# Autodesk Inventor assembly: Extruder Assembly
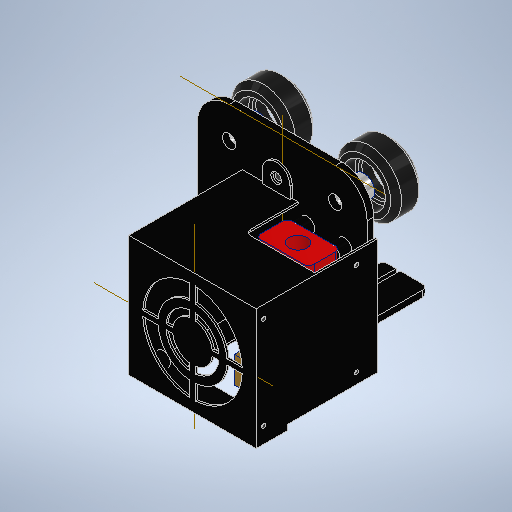
[picture p0: Inventor's stored thumbnail of the model, 512x512]
Saved by Autodesk Inventor 2025.2 (Build 292293000, 293)
## iProperties
Created: 2025-03-12
Part Number: Extruder Assembly
Document SubType Name: Assembly
Designer: MAL16204
Author: MAL16204
## Documents named in this file (7)
- C:\Users\rdmal\OneDrive - Pennsylvania Western University\Spring 2025\MECH 2400\CAD Projects\Final Project\Extruder Assembly.iam
- C:\Users\rdmal\OneDrive - Pennsylvania Western University\Spring 2025\MECH 2400\CAD Projects\Final Project\Hotend.ipt
- C:\Users\rdmal\OneDrive - Pennsylvania Western University\Spring 2025\MECH 2400\CAD Projects\Final Project\Nozzle 0.4mm.ipt
- C:\Users\rdmal\OneDrive - Pennsylvania Western University\Spring 2025\MECH 2400\CAD Projects\Final Project\Extruder Plate.ipt
- C:\Users\rdmal\OneDrive - Pennsylvania Western University\Spring 2025\MECH 2400\CAD Projects\Final Project\Spacers for Rollers.ipt
- C:\Users\rdmal\OneDrive - Pennsylvania Western University\Spring 2025\MECH 2400\CAD Projects\Final Project\Rollers.ipt
- C:\Users\rdmal\OneDrive - Pennsylvania Western University\Spring 2025\MECH 2400\CAD Projects\Final Project\Fan Cover.ipt
## Components (10 placed, 6 different names)
1. Hotend:1 — Cylindrical:1, Rigid:1
2. Nozzle 0.4mm:1 — Cylindrical:1
3. Extruder Plate:1 — Rigid:1, Rotational:1, Rotational:2, Rotational:3, Rigid:2
4. Spacers for Rollers:1 — Rotational:3, Rotational:6
5. Spacers for Rollers:2 — Rotational:1, Rotational:4
6. Spacers for Rollers:3 — Rotational:2, Rotational:5
7. Rollers:1 — Rotational:5
8. Rollers:2 — Rotational:6
9. Rollers:3 — Rotational:4
10. Fan Cover:1 — Rigid:2
## Relationships (9: RevoluteJoint 6, WeldJoint 2, CylindricalJoint 1)
- Cylindrical:1: Hotend:1 ↔ Nozzle 0.4mm:1
- Rigid:1 [WeldJoint]: Hotend:1 ↔ Extruder Plate:1
- Rotational:1 [RevoluteJoint]: Extruder Plate:1 ↔ Spacers for Rollers:2
- Rotational:2 [RevoluteJoint]: Extruder Plate:1 ↔ Spacers for Rollers:3
- Rotational:3 [RevoluteJoint]: Extruder Plate:1 ↔ Spacers for Rollers:1
- Rotational:4 [RevoluteJoint]: Spacers for Rollers:2 ↔ Rollers:3
- Rotational:5 [RevoluteJoint]: Spacers for Rollers:3 ↔ Rollers:1
- Rotational:6 [RevoluteJoint]: Spacers for Rollers:1 ↔ Rollers:2
- Rigid:2 [WeldJoint]: Extruder Plate:1 ↔ Fan Cover:1
